# Autodesk Inventor assembly: TOTEM_Slider_Y
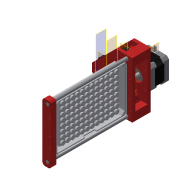
[picture p0: Inventor's stored thumbnail of the model, 180x180]
Saved by Autodesk Inventor 2019.4 (Build 234330000, 330)
## iProperties
Created: 2021-10-10
Part Number: TOTEM_Slider_Y
Document SubType Name: Assembly
Designer: diederichbenedict
Author: diederichbenedict
## Documents named in this file (7)
- C:\Users\diederichbenedict\Dropbox\Dokumente\Promotion\PROJECTS\UC2\02_CAD\INVENTOR\uc2_v3\TOTEM_Slider_Y.iam
- C:\Users\diederichbenedict\Dropbox\Dokumente\Promotion\PROJECTS\UC2\02_CAD\INVENTOR\uc2_v3\TOTEM_Base_Slide_y_20mmrod.ipt
- C:\Users\diederichbenedict\Dropbox\Dokumente\Promotion\PROJECTS\UC2\02_CAD\INVENTOR\uc2_v3\00_Thorlabs_Rod_6mm.ipt
- C:\Users\diederichbenedict\Dropbox\Dokumente\Promotion\PROJECTS\UC2\02_CAD\INVENTOR\uc2_v3\Neje_Base_Slide_y_stop.ipt
- C:\Users\diederichbenedict\Dropbox\Dokumente\Promotion\PROJECTS\UC2\02_CAD\INVENTOR\uc2_v3\00_MTP_96-welplate.ipt
- C:\Users\diederichbenedict\Dropbox\Dokumente\Promotion\PROJECTS\UC2\02_CAD\INVENTOR\uc2_v3\00_NEMA17.ipt
- C:\Users\diederichbenedict\Dropbox\Dokumente\Promotion\PROJECTS\UC2\02_CAD\INVENTOR\uc2_v3\Neje_Rolls.ipt
## Components (10 placed, 6 different names)
1. TOTEM_Base_Slide_y_20mmrod:1 — Insert:1, Angle:1, Insert:4, Insert:5, Insert:6, Insert:7, Insert:8, Insert:9, Insert:10
2. TOTEM_Base_Slide_y_20mmrod:2 — Insert:1, Angle:1, Flush:3, Flush:4
3. 00_Thorlabs_Rod_6mm:2 — Insert:6
4. Neje_Base_Slide_y_stop:1 — Mate:1
5. 00_MTP_96-welplate:1
6. 00_NEMA17:1 — Insert:4, Insert:5
7. 00_Thorlabs_Rod_6mm:3 — Insert:7, Mate:1
8. Neje_Rolls:1 — Insert:10
9. Neje_Rolls:2 — Insert:9
10. Neje_Rolls:3 — Insert:8
## Relationships (16: Insert 9, Flush 4, Angle 1, Mate 1, Symmetry 1)
- Insert:1: TOTEM_Base_Slide_y_20mmrod:1 ↔ TOTEM_Base_Slide_y_20mmrod:2
- Angle:1 (180 deg): TOTEM_Base_Slide_y_20mmrod:1 ↔ TOTEM_Base_Slide_y_20mmrod:2
- [Insert]: 00_Thorlabs_Rod_6mm:2 ↔ Neje_Base_Slide_y_stop:1
- [Flush] (9 mm): Neje_Base_Slide_y_stop:1 ↔ 00_MTP_96-welplate:1
- [Flush] (11.5 mm): Neje_Base_Slide_y_stop:1 ↔ 00_MTP_96-welplate:1
- Insert:4: TOTEM_Base_Slide_y_20mmrod:1 ↔ 00_NEMA17:1
- Insert:5: TOTEM_Base_Slide_y_20mmrod:1 ↔ 00_NEMA17:1
- Insert:6: TOTEM_Base_Slide_y_20mmrod:1 ↔ 00_Thorlabs_Rod_6mm:2
- Insert:7: TOTEM_Base_Slide_y_20mmrod:1 ↔ 00_Thorlabs_Rod_6mm:3
- Mate:1: Neje_Base_Slide_y_stop:1 ↔ 00_Thorlabs_Rod_6mm:3
- Insert:8: TOTEM_Base_Slide_y_20mmrod:1 ↔ Neje_Rolls:3
- Insert:9: TOTEM_Base_Slide_y_20mmrod:1 ↔ Neje_Rolls:2
- Insert:10: TOTEM_Base_Slide_y_20mmrod:1 ↔ Neje_Rolls:1
- Flush:3 (-26 mm): TOTEM_Base_Slide_y_20mmrod:2
- Flush:4 (-8 mm): TOTEM_Base_Slide_y_20mmrod:2
- Symmetry:1
